# Autodesk Inventor assembly: mg996r 3mm foot
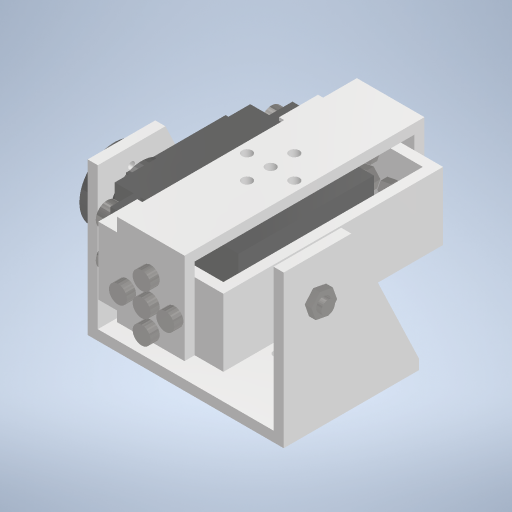
[picture p0: Inventor's stored thumbnail of the model, 512x512]
Saved by Autodesk Inventor 2023 (Build 270158000, 158)
## iProperties
Created: 2022-06-29
Part Number: mg996r 3mm foot
Document SubType Name: Assembly
Designer: isamu
Author: isamu
## iProperties of the stored document servo frame mg996r008.ipt
Created: 2022-06-29
Part Number: servo frame mg996r008
Material: Generic
Document SubType Name: Modeling
Designer: isamu
Density: 1 g/cm^3
Appearance: Default
Author: isamu
## iProperties of the stored document servo frame mg996 foot.iam
Created: 2022-06-29
Part Number: servo frame mg996 foot
Description: FreeCAD Model
Document SubType Name: Assembly
Designer: isamu
Authority: Unknown
Title: Open CASCADE Shape Model
Author: Author
Sending System: FreeCAD
Preprocessor: Open CASCADE STEP processor 7.5
## Documents named in this file (6)
- **D:\personal_projects\robot\inventor\mg996r 3mm foot.iam*LocalDocs*xAaaaqtcaAaaaaaaaAaaaqthnDe*servo frame mg996r008.ipt
- **D:\personal_projects\robot\inventor\mg996r 3mm foot.iam*LocalDocs*xAaaaq0baAaaaaaaaAaaaauutDc*servo frame mg996 foot.iam
- D:\personal_projects\robot\inventor\mg996r 3mm foot.iam
- D:\personal_projects\robot\inventor\base mg996r 3mm with top.iam
- D:\personal_projects\robot\exports\frames\m4 nuts.ipt
- D:\personal_projects\robot\exports\frames\servo frame mg996 foot.step
## Components (3 placed, 3 different names)
1. base mg996r 3mm with top:1 [sub-assembly] — Mate:1, Mate:2, Mate:3
2. servo frame mg996 foot:1 [sub-assembly] — Mate:1, Mate:2, Mate:3, Insert:1
3. m4 nuts:1 — Insert:1
## Relationships (4: Mate 3, Insert 1)
- Mate:1: base mg996r 3mm with top:1 ↔ servo frame mg996 foot:1
- Mate:2: base mg996r 3mm with top:1 ↔ servo frame mg996 foot:1
- Mate:3: base mg996r 3mm with top:1 ↔ servo frame mg996 foot:1
- Insert:1: servo frame mg996 foot:1 ↔ m4 nuts:1
